# Autodesk Inventor assembly: Hitec Servo
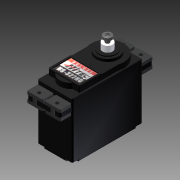
[picture p0: Inventor's stored thumbnail of the model, 180x180]
Saved by Autodesk Inventor 2012 (Build 160160000, 160)
## iProperties
Shininess: 64.0
Length Units: 11269
Angle Units: 11279
Time Units: 11290
Mass Units: 11283
Length Display Precision: 3
Angle Display Precision: 2
Compacted: True
Created: 2006-01-16
Part Number: Hitec Servo
Document SubType Name: Assembly
Designer: Ed Sparks
Density: 0.0
Volumn: 0.0
Area: 0.0
PropertySet Name: Model Information
Control State: 0
Master: False
Checked Out: False
Author: Ed Sparks
## Documents named in this file (5)
- C:\Users\Bryce\Dropbox\Rebound Rumble 2012\Independant Swerves\Imported Components\Hitec Servo.iam
- C:\Users\Bryce\Dropbox\Rebound Rumble 2012\Independant Swerves\Imported Components\Hitec Servo.ipt
- C:\Users\Bryce\Dropbox\Rebound Rumble 2012\Independant Swerves\Imported Components\Servo Screw.ipt
- C:\Users\Bryce\Dropbox\Rebound Rumble 2012\Independant Swerves\Imported Components\Screw2.ipt
- C:\Users\Bryce\Dropbox\Rebound Rumble 2012\Independant Swerves\Imported Components\Servo Isolation Mounts.ipt
## Components (10 placed, 4 different names)
1. Hitec Servo:1 — Mate:1, Mate:2, Mate:5, Mate:6, Mate:7, Mate:8, Mate:9, Mate:10
2. Screw2:1
3. Servo Screw:1 — Mate:1, Mate:2
4. Servo Screw:2
5. Servo Screw:3
6. Servo Screw:4
7. Servo Isolation Mounts:2 — Mate:8, Mate:9, Mate:10
8. Servo Isolation Mounts:1 — Mate:5, Mate:6, Mate:7
9. Servo Isolation Mounts:3
10. Servo Isolation Mounts:4
## Component patterns: Screws (4 elements), Isolation Mounts (2 elements)
## Relationships (8: Mate 8)
- Mate:1: Hitec Servo:1 ↔ Servo Screw:1
- Mate:2: Hitec Servo:1 ↔ Servo Screw:1
- Mate:5: Hitec Servo:1 ↔ Servo Isolation Mounts:1
- Mate:6: Hitec Servo:1 ↔ Servo Isolation Mounts:1
- Mate:7: Hitec Servo:1 ↔ Servo Isolation Mounts:1
- Mate:8: Hitec Servo:1 ↔ Servo Isolation Mounts:2
- Mate:9: Hitec Servo:1 ↔ Servo Isolation Mounts:2
- Mate:10: Hitec Servo:1 ↔ Servo Isolation Mounts:2
